# Autodesk Inventor assembly: Microdrive_Compact_withCase_Body
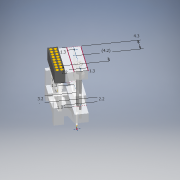
[picture p0: Inventor's stored thumbnail of the model, 180x180]
Saved by Autodesk Inventor 2020 (Build 240168000, 168)
## iProperties
Created: 2019-11-04
Part Number: Microdrive_Compact_withCase_Body
Document SubType Name: Assembly
Designer: Knowblesse
Author: Knowblesse
## Documents named in this file (14)
- C:\VCF\Microdrive\Compact\Microdrive_Compact.iam
- C:\VCF\Microdrive\Compact\PCB.ipt
- C:\VCF\Microdrive\Compact\Millmax.ipt
- C:\VCF\Microdrive\Compact\Body.ipt
- C:\VCF\Microdrive\Compact\Bot.ipt
- C:\VCF\Microdrive\Compact\Screw.ipt
- C:\VCF\Microdrive\Compact\Top.ipt
- C:\VCF\Microdrive\Compact\Nut.ipt
- C:\VCF\Microdrive\Compact\23G_Pillar.ipt
- C:\VCF\Microdrive\Compact\23G_Holder.ipt
- C:\VCF\Microdrive\Compact\Polyimide.ipt
- C:\VCF\Microdrive\Compact\Tetrode.ipt
- C:\VCF\Microdrive\Compact\Case.ipt
- C:\VCF\Microdrive\Compact\Case_Cover.ipt
## Components (14 placed, 13 different names)
1. Body:1 — 강체:2, 메이트:1, 회전:5, 회전:6, 강체:5
2. Bot:1 — 메이트:2, 메이트:3, 회전:8
3. Screw:1 — 회전:1, 메이트:1, 메이트:2
4. Top:1 — 회전:1, 회전:2, 회전:4, 회전:7
5. Millmax:1 — 강체:1
6. Nut:1 — 회전:2
7. PCB:1 — 강체:1, 강체:2
8. 23G_Pillar:1 — 회전:4, 회전:5
9. 23G_Pillar:2 — 회전:6, 회전:7, 메이트:3
10. 23G_Holder:1 — 회전:8, 강체:4
11. Polyimide:1 — 강체:3, 강체:4
12. Tetrode:1 — 강체:3
13. Case:1 — 강체:5, 강체:6
14. Case_Cover:1 — 강체:6
## Relationships (16: RevoluteJoint 7, WeldJoint 6, Mate 3)
- 강체:1 [WeldJoint]: Millmax:1 ↔ PCB:1
- 강체:2 [WeldJoint]: Body:1 ↔ PCB:1
- 회전:1 [RevoluteJoint]: Screw:1 ↔ Top:1
- 회전:2 [RevoluteJoint]: Top:1 ↔ Nut:1
- 메이트:1 [Mate]: Body:1 ↔ Screw:1
- 메이트:2 [Mate]: Bot:1 ↔ Screw:1
- 회전:4 [RevoluteJoint]: Top:1 ↔ 23G_Pillar:1
- 회전:5 [RevoluteJoint]: Body:1 ↔ 23G_Pillar:1
- 회전:6 [RevoluteJoint]: Body:1 ↔ 23G_Pillar:2
- 회전:7 [RevoluteJoint]: Top:1 ↔ 23G_Pillar:2
- 메이트:3 [Mate]: Bot:1 ↔ 23G_Pillar:2
- 회전:8 [RevoluteJoint] (0.5 mm): Bot:1 ↔ 23G_Holder:1
- 강체:3 [WeldJoint] (-1 mm): Polyimide:1 ↔ Tetrode:1
- 강체:4 [WeldJoint] (0.5 mm): 23G_Holder:1 ↔ Polyimide:1
- 강체:5 [WeldJoint]: Body:1 ↔ Case:1
- 강체:6 [WeldJoint]: Case:1 ↔ Case_Cover:1
